# Autodesk Inventor assembly: Weapon (Motor-Side Pulley)
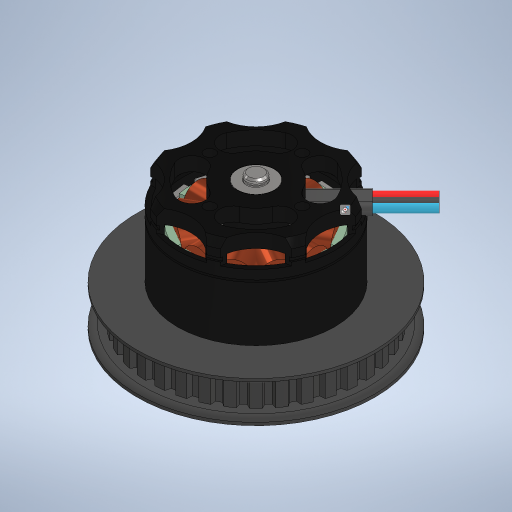
[picture p0: Inventor's stored thumbnail of the model, 512x512]
Saved by Autodesk Inventor 2023 (Build 270158000, 158)
## iProperties
Created: 2022-05-21
Part Number: Weapon (Motor-Side Pulley)
Document SubType Name: Assembly
Designer: Nathan Cai
Mass: 163.794 g
Surface Area: 513.523 cm^2
Volume: 53.858 cm^3
Density: 3.04123 g/cm^3
Author: Nathan Cai
## Documents named in this file (4)
- E:\Documents\Inventor\0.3rd Lawette - V3.3\Weapon (Motor-Side Pulley).iam
- E:\Documents\Inventor\0.3rd Lawette - V3.3\XL Pulley 36T .375in Wd.ipt
- E:\Documents\Inventor\0.3rd Lawette - V3.3\Aerosky MC4230 630KV\Aerosky_MC4230_630KV.iam
- E:\Documents\Inventor\0.3rd Lawette - V3.3\Interface Plate.ipt
## Components (3 placed, 3 different names)
1. XL Pulley 36T .375in Wd:1 — Mate:1, Mate:5, Mate:6
2. Aerosky_MC4230_630KV:1 [sub-assembly] — Mate:1, Mate:3, Mate:4, Mate:5
3. Interface Plate:1 — Mate:3, Mate:4, Mate:6
## Relationships (5: Mate 5)
- Mate:1: XL Pulley 36T .375in Wd:1 ↔ Aerosky_MC4230_630KV:1
- Mate:3: Aerosky_MC4230_630KV:1 ↔ Interface Plate:1
- Mate:4: Aerosky_MC4230_630KV:1 ↔ Interface Plate:1
- Mate:5 (-34.925 mm): XL Pulley 36T .375in Wd:1 ↔ Aerosky_MC4230_630KV:1
- Mate:6: XL Pulley 36T .375in Wd:1 ↔ Interface Plate:1
